# Autodesk Inventor assembly: edf_drone_v1
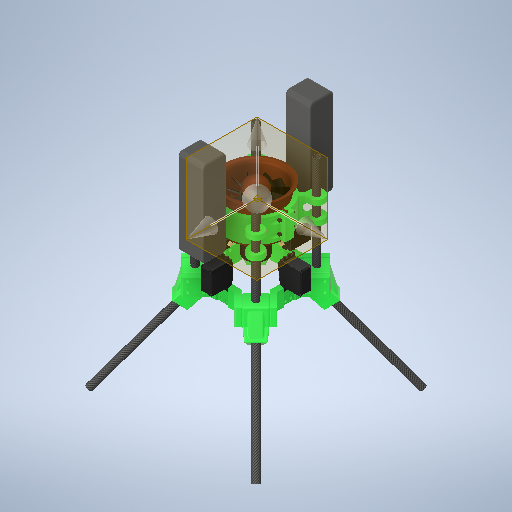
[picture p0: Inventor's stored thumbnail of the model, 512x512]
Saved by Autodesk Inventor 2026.2 (Build 302298010, 298A)
## iProperties
Created: 2026-03-12
Part Number: edf_drone_v1
Document SubType Name: Assembly
Designer: tngzj
Mass: 2553.69 g
Surface Area: 4575.14 cm^2
Volume: 1535.13 cm^3
Density: 1.6635 g/cm^3
Author: tngzj
## Documents named in this file (10)
- C:\Transformer-rl-retro-propulsion\CAD\EDF Drone v1\edf_drone_v1.iam
- C:\Transformer-rl-retro-propulsion\CAD\EDF Drone v1\Fan\fms 90mm edf.iam
- C:\Transformer-rl-retro-propulsion\CAD\EDF Drone v1\Structure\Carbon Fiber Tube 12mm x 10mm.ipt
- C:\Transformer-rl-retro-propulsion\CAD\EDF Drone v1\Structure\EDF Mount v1.ipt
- C:\Users\tngzj\OneDrive\Documents\Inventor\Content Center Files\R2026\en-US\ISO 14580_2011(E)\ISO 14580 M3.5x25-4.8.ipt
- C:\Users\tngzj\OneDrive\Documents\Inventor\Content Center Files\R2026\en-US\ISO 4032(2)\ISO 4032 - M3.5 - ISO.ipt
- C:\Transformer-rl-retro-propulsion\CAD\EDF Drone v1\Servo\MG996R Servo.ipt
- C:\Transformer-rl-retro-propulsion\CAD\EDF Drone v1\Structure\Leg Adaptor.ipt
- C:\Transformer-rl-retro-propulsion\CAD\EDF Drone v1\Battery\OVONIC 6S LiPo Battery.ipt
- C:\Transformer-rl-retro-propulsion\CAD\EDF Drone v1\Structure\Cross Links.ipt
## Components (33 placed, 9 different names)
1. fms 90mm edf:1 [sub-assembly] — Mate:10, Mate:11, Angle:3, Mate:13, Flush:2, Mate:14, Angle:4, Mate:86
2. EDF Mount v1:1 — Flush:2, Mate:14, Flush:3, Angle:4, Mate:19, Mate:20, Mate:21, Mate:23, Mate:24, Mate:25, Mate:27, Mate:28, Mate:31, Mate:32, Mate:33, Mate:35, Mate:36, Mate:37, Flush:8, Flush:14
3. EDF Mount v1:2 — Mate:13, Flush:3, Mate:22, Mate:26, Mate:29, Mate:30, Mate:34, Mate:38
4. Screw ISO 14580:2011(E) M3.5x25-4.8:2 — Mate:35, Mate:36
5. ISO 4032 M3.5:2 — Mate:37, Mate:38
6. Screw ISO 14580:2011(E) M3.5x25-4.8:3 — Mate:19, Mate:20
7. ISO 4032 M3.5:3 — Mate:21, Mate:22
8. Screw ISO 14580:2011(E) M3.5x25-4.8:4 — Mate:23, Mate:24
9. ISO 4032 M3.5:4 — Mate:25, Mate:26
10. Screw ISO 14580:2011(E) M3.5x25-4.8:5 — Mate:31, Mate:32
11. ISO 4032 M3.5:5 — Mate:33, Mate:34
12. Carbon Fiber Tube 12mm x 10mm:2 — Mate:28, Flush:4, Flush:5, Flush:8, Mate:50, Mate:54
13. Carbon Fiber Tube 12mm x 10mm:3 — Mate:29, Flush:7, Mate:39, Mate:40
14. Carbon Fiber Tube 12mm x 10mm:4 — Mate:30, Flush:6, Mate:49, Mate:52
15. Carbon Fiber Tube 12mm x 10mm:1 — Mate:27, Flush:4, Flush:5, Flush:6, Flush:7, Mate:51, Mate:53
16. MG996R Servo:1 — Mate:74, Mate:67, Mate:75
17. MG996R Servo:2 — Mate:68, Mate:78, Mate:79
18. MG996R Servo:3 — Mate:71, Mate:77, Mate:80
19. MG996R Servo:4 — Mate:73, Mate:76, Mate:81
20. Leg Adaptor:1 — Mate:39, Mate:40, Angle:5, Mate:41, Mate:42, Mate:55, Mate:56, Mate:57
21. Carbon Fiber Tube 12mm x 10mm:5 — Mate:41, Mate:42
22. Leg Adaptor:2 — Mate:49, Angle:6, Mate:52, Mate:58, Mate:59, Mate:60, Flush:9
23. Carbon Fiber Tube 12mm x 10mm:6
24. Leg Adaptor:3 — Mate:51, Mate:53, Angle:7, Mate:61, Mate:62, Mate:63
25. Carbon Fiber Tube 12mm x 10mm:7
26. Leg Adaptor:4 — Mate:50, Mate:54, Angle:8, Mate:64, Mate:65, Mate:66
27. Carbon Fiber Tube 12mm x 10mm:8
28. Cross Links:1 — Mate:55, Mate:56, Mate:57, Mate:68, Mate:78, Mate:79
29. Cross Links:2 — Mate:61, Mate:62, Mate:63, Mate:73, Mate:76, Mate:81
30. Cross Links:3 — Mate:58, Mate:59, Mate:60, Flush:9, Mate:71, Mate:77, Mate:80
31. Cross Links:4 — Mate:64, Mate:65, Mate:66, Mate:74, Mate:67, Mate:75
32. OVONIC 6S LiPo Battery:3 — Flush:11, Flush:13, Mate:84, Mate:85, Mate:86, Flush:14
33. OVONIC 6S LiPo Battery:1 — Flush:11, Flush:13, Mate:84
## Relationships (84: Mate 67, Flush 11, Angle 6)
- Mate:10: fms 90mm edf:1
- Mate:11: fms 90mm edf:1
- Angle:3 (0 deg): fms 90mm edf:1
- Mate:13: fms 90mm edf:1 ↔ EDF Mount v1:2
- Flush:2: fms 90mm edf:1 ↔ EDF Mount v1:1
- Mate:14: fms 90mm edf:1 ↔ EDF Mount v1:1
- Flush:3: EDF Mount v1:1 ↔ EDF Mount v1:2
- Angle:4 (-180 deg): fms 90mm edf:1 ↔ EDF Mount v1:1
- Mate:19: EDF Mount v1:1 ↔ Screw ISO 14580:2011(E) M3.5x25-4.8:3
- Mate:20: EDF Mount v1:1 ↔ Screw ISO 14580:2011(E) M3.5x25-4.8:3
- Mate:21: EDF Mount v1:1 ↔ ISO 4032 M3.5:3
- Mate:22: EDF Mount v1:2 ↔ ISO 4032 M3.5:3
- Mate:23: EDF Mount v1:1 ↔ Screw ISO 14580:2011(E) M3.5x25-4.8:4
- Mate:24: EDF Mount v1:1 ↔ Screw ISO 14580:2011(E) M3.5x25-4.8:4
- Mate:25: EDF Mount v1:1 ↔ ISO 4032 M3.5:4
- Mate:26: EDF Mount v1:2 ↔ ISO 4032 M3.5:4
- Mate:27: EDF Mount v1:1 ↔ Carbon Fiber Tube 12mm x 10mm:1
- Mate:28: EDF Mount v1:1 ↔ Carbon Fiber Tube 12mm x 10mm:2
- Mate:29: EDF Mount v1:2 ↔ Carbon Fiber Tube 12mm x 10mm:3
- Mate:30: EDF Mount v1:2 ↔ Carbon Fiber Tube 12mm x 10mm:4
- Mate:31: EDF Mount v1:1 ↔ Screw ISO 14580:2011(E) M3.5x25-4.8:5
- Mate:32: EDF Mount v1:1 ↔ Screw ISO 14580:2011(E) M3.5x25-4.8:5
- Mate:33: EDF Mount v1:1 ↔ ISO 4032 M3.5:5
- Mate:34: EDF Mount v1:2 ↔ ISO 4032 M3.5:5
- Mate:35: EDF Mount v1:1 ↔ Screw ISO 14580:2011(E) M3.5x25-4.8:2
- Mate:36: EDF Mount v1:1 ↔ Screw ISO 14580:2011(E) M3.5x25-4.8:2
- Mate:37: EDF Mount v1:1 ↔ ISO 4032 M3.5:2
- Mate:38: EDF Mount v1:2 ↔ ISO 4032 M3.5:2
- Flush:4: Carbon Fiber Tube 12mm x 10mm:2 ↔ Carbon Fiber Tube 12mm x 10mm:1
- Flush:5: Carbon Fiber Tube 12mm x 10mm:2 ↔ Carbon Fiber Tube 12mm x 10mm:1
- Flush:6: Carbon Fiber Tube 12mm x 10mm:4 ↔ Carbon Fiber Tube 12mm x 10mm:1
- Flush:7: Carbon Fiber Tube 12mm x 10mm:3 ↔ Carbon Fiber Tube 12mm x 10mm:1
- Mate:39: Carbon Fiber Tube 12mm x 10mm:3 ↔ Leg Adaptor:1
- Flush:8 (-100 mm): EDF Mount v1:1 ↔ Carbon Fiber Tube 12mm x 10mm:2
- Mate:40: Carbon Fiber Tube 12mm x 10mm:3 ↔ Leg Adaptor:1
- Angle:5 (45 deg): Leg Adaptor:1
- Mate:41: Leg Adaptor:1 ↔ Carbon Fiber Tube 12mm x 10mm:5
- Mate:42: Leg Adaptor:1 ↔ Carbon Fiber Tube 12mm x 10mm:5
- [Mate]: Leg Adaptor:2 ↔ Carbon Fiber Tube 12mm x 10mm:6
- [Mate]: Leg Adaptor:2 ↔ Carbon Fiber Tube 12mm x 10mm:6
- [Mate]: Leg Adaptor:3 ↔ Carbon Fiber Tube 12mm x 10mm:7
- [Mate]: Leg Adaptor:3 ↔ Carbon Fiber Tube 12mm x 10mm:7
- [Mate]: Leg Adaptor:4 ↔ Carbon Fiber Tube 12mm x 10mm:8
- [Mate]: Leg Adaptor:4 ↔ Carbon Fiber Tube 12mm x 10mm:8
- Mate:49: Carbon Fiber Tube 12mm x 10mm:4 ↔ Leg Adaptor:2
- Mate:50: Carbon Fiber Tube 12mm x 10mm:2 ↔ Leg Adaptor:4
- Mate:51: Carbon Fiber Tube 12mm x 10mm:1 ↔ Leg Adaptor:3
- Angle:6 (45 deg): Leg Adaptor:2
- Mate:52: Carbon Fiber Tube 12mm x 10mm:4 ↔ Leg Adaptor:2
- Mate:53: Carbon Fiber Tube 12mm x 10mm:1 ↔ Leg Adaptor:3
- Mate:54: Carbon Fiber Tube 12mm x 10mm:2 ↔ Leg Adaptor:4
- Angle:7 (-135 deg): Leg Adaptor:3
- Angle:8 (45 deg): Leg Adaptor:4
- Mate:55: Leg Adaptor:1 ↔ Cross Links:1
- Mate:56: Leg Adaptor:1 ↔ Cross Links:1
- Mate:57: Leg Adaptor:1 ↔ Cross Links:1
- Mate:58: Leg Adaptor:2 ↔ Cross Links:3
- Mate:59: Leg Adaptor:2 ↔ Cross Links:3
- Mate:60: Leg Adaptor:2 ↔ Cross Links:3
- Flush:9: Leg Adaptor:2 ↔ Cross Links:3
- Mate:61: Leg Adaptor:3 ↔ Cross Links:2
- Mate:62: Leg Adaptor:3 ↔ Cross Links:2
- Mate:63: Leg Adaptor:3 ↔ Cross Links:2
- Mate:64: Leg Adaptor:4 ↔ Cross Links:4
- Mate:65: Leg Adaptor:4 ↔ Cross Links:4
- Mate:66: Leg Adaptor:4 ↔ Cross Links:4
- Mate:74: MG996R Servo:1 ↔ Cross Links:4
- Mate:67: MG996R Servo:1 ↔ Cross Links:4
- Mate:68: MG996R Servo:2 ↔ Cross Links:1
- Mate:71: MG996R Servo:3 ↔ Cross Links:3
- Mate:73: MG996R Servo:4 ↔ Cross Links:2
- Mate:75: MG996R Servo:1 ↔ Cross Links:4
- Mate:76: MG996R Servo:4 ↔ Cross Links:2
- Mate:77: MG996R Servo:3 ↔ Cross Links:3
- Mate:78: MG996R Servo:2 ↔ Cross Links:1
- Mate:79: MG996R Servo:2 ↔ Cross Links:1
- Mate:80: MG996R Servo:3 ↔ Cross Links:3
- Mate:81: MG996R Servo:4 ↔ Cross Links:2
- Flush:11: OVONIC 6S LiPo Battery:3 ↔ OVONIC 6S LiPo Battery:1
- Flush:13: OVONIC 6S LiPo Battery:3 ↔ OVONIC 6S LiPo Battery:1
- Mate:84 (150 mm): OVONIC 6S LiPo Battery:3 ↔ OVONIC 6S LiPo Battery:1
- Mate:85: OVONIC 6S LiPo Battery:3
- Mate:86 (75 mm): fms 90mm edf:1 ↔ OVONIC 6S LiPo Battery:3
- Flush:14: EDF Mount v1:1 ↔ OVONIC 6S LiPo Battery:3
## Named parameters: d61_d60 = 0 mm, d62_d59 = 0 mm, d63_d60 = 0 mm, d64_d59 = 0 mm, d65_d60 = 0 mm, d66_d59 = 0 mm
